# Autodesk Inventor assembly: assemble_ver5
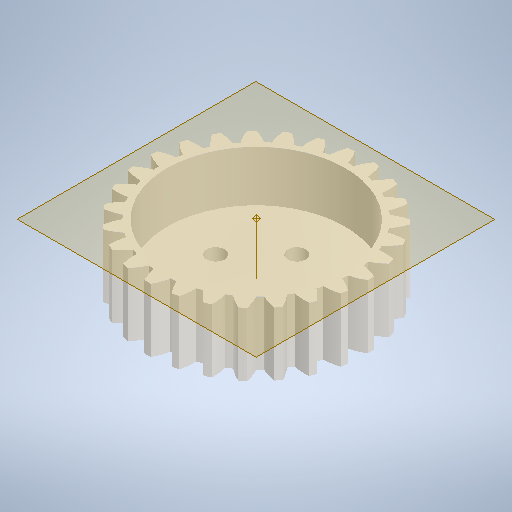
[picture p0: Inventor's stored thumbnail of the model, 512x512]
Saved by Autodesk Inventor 2025 (Build 290162000, 162)
## iProperties
Created: 2025-12-09
Part Number: assemble_ver5
Document SubType Name: Assembly
Designer: Admin
Author: Admin
## Documents named in this file (2)
- C:\Users\sum89\OneDrive\Рабочий стол\Ring\Model\assemble_ver5.iam
- C:\Users\sum89\OneDrive\Рабочий стол\Ring\Model\assemble_ver5\Мастер проектирования\Цилиндрическое зубчатое зацепление1.iam
## Components (1 placed, 1 different names)
1. Цилиндрическое зубчатое зацепление:1 [sub-assembly] — Совмещение:1, Совмещение:2, Совмещение:3, Угол:1
## Relationships (6: Mate 5, Angle 1)
- Совмещение:1 [Mate]: Цилиндрическое зубчатое зацепление:1
- Совмещение:2 [Mate]: Цилиндрическое зубчатое зацепление:1
- Совмещение:3 [Mate]: Цилиндрическое зубчатое зацепление:1
- Совмещение:4 [Mate]
- Совмещение:5 [Mate]
- Угол:1 [Angle] (0 deg): Цилиндрическое зубчатое зацепление:1
